# Autodesk Inventor assembly: Cylinder
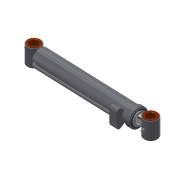
[picture p0: Inventor's stored thumbnail of the model, 180x180]
Saved by Autodesk Inventor 2022 Beta2 (Build 260130000, 130) ContinuousBuild 0
## iProperties
Shininess: 0.0
Length Units: 11269
Angle Units: 11279
Time Units: 11290
Mass Units: 11283
Length Display Precision: 3
Angle Display Precision: 2
Part Number: Cylinder
Description: Cylinder 63/32-350 complete
Document SubType Name: Assembly
Designer: Joe M
Engineer: Joe M
Created: 2016-01-21
Density: 0.0
Volume: 0.0
Area: 0.0
PropertySet Name: Model Information
Control State: 0
Master: False
Checked Out: False
Title: Cylinder 63/32-350 komplett
Author: Joe M
## Documents named in this file (3)
- C:\Autodesk Inventor 2021 Intro Practice Files\BOM\Cylinder.iam
- C:\Autodesk Inventor 2021 Intro Practice Files\BOM\Cylinder Tube.iam
- C:\Autodesk Inventor 2021 Intro Practice Files\BOM\Cylinder Piston Rod.iam
## Components (2 placed, 2 different names)
1. Cylinder Tube:1 [sub-assembly] — Mate:1, Angle:1, Stroke
2. Cylinder Piston Rod:1 [sub-assembly] — Mate:1, Angle:1, Stroke
## Relationships (3: Mate 2, Angle 1)
- Mate:1: Cylinder Tube:1 ↔ Cylinder Piston Rod:1
- Angle:1 (0 deg): Cylinder Tube:1 ↔ Cylinder Piston Rod:1
- Stroke [Mate]: Cylinder Tube:1 ↔ Cylinder Piston Rod:1
